# Autodesk Inventor assembly: 車体
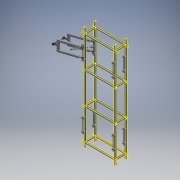
[picture p0: Inventor's stored thumbnail of the model, 180x180]
Saved by Autodesk Inventor 2018 (Build 220112000, 112)
## iProperties
Created: 2017-09-11
Part Number: 車体
Material: 一般
Document SubType Name: Assembly
Designer: mura5
Author: mura5
## Documents named in this file (8)
- C:\Users\Kenta\Documents\workspace\rbbr\cart\シャーシ改でアッカーマン検討\車体.iam
- C:\Users\Kenta\Documents\workspace\rbbr\cart\シャーシ改でアッカーマン検討\Pipe1.ipt
- C:\Users\Kenta\Documents\workspace\rbbr\cart\シャーシ改でアッカーマン検討\Pipe2.ipt
- C:\Users\Kenta\Documents\workspace\rbbr\cart\シャーシ改でアッカーマン検討\Pipe3.ipt
- C:\Users\Kenta\Documents\workspace\rbbr\cart\シャーシ改でアッカーマン検討\Pipe4.ipt
- C:\Users\Kenta\Documents\workspace\rbbr\cart\シャーシ\飛び出す奴上.iam
- C:\Users\Kenta\Documents\workspace\rbbr\cart\A.iam
- C:\Users\Kenta\Documents\workspace\rbbr\cart\スプリング.iam
## Components (31 placed, 7 different names)
1. Pipe1:1 — 回転:1, 角度:1, 回転:3, 角度:3, メイト:1, フラッシュ:1, フラッシュ:2, メイト:3, メイト:13, メイト:14, メイト:16, フラッシュ:5, メイト:18, フラッシュ:10, メイト:20, メイト:30, メイト:43, 角度:9
2. Pipe2:1 — 回転:1, 回転:2, 角度:1, 角度:2, メイト:2, フラッシュ:8, フラッシュ:9, 角度:5, メイト:31, メイト:37
3. Pipe1:2 — 回転:2, 角度:2, メイト:7, メイト:10, メイト:12, フラッシュ:7, メイト:17, メイト:35, 角度:7, メイト:45, 角度:11
4. Pipe2:2 — 回転:3, 角度:3, メイト:4, メイト:5, メイト:6, メイト:8, フラッシュ:12, メイト:48, メイト:50
5. Pipe3:1 — メイト:1, フラッシュ:1, メイト:2, メイト:11, フラッシュ:4, フラッシュ:6
6. Pipe3:2 — フラッシュ:2, メイト:3, メイト:4, メイト:9, フラッシュ:3, メイト:15
7. Pipe4:1 — メイト:5, フラッシュ:11, メイト:19, メイト:20, フラッシュ:12, フラッシュ:13
8. Pipe4:2 — メイト:6, メイト:7, メイト:8
9. Pipe4:3 — メイト:13, メイト:14, メイト:15
10. Pipe4:4 — メイト:16, フラッシュ:5, フラッシュ:6
11. Pipe4:5 — メイト:11, メイト:12, フラッシュ:4, フラッシュ:15
12. Pipe4:6 — メイト:9, メイト:10, フラッシュ:3, フラッシュ:16
13. Pipe4:7 — メイト:18, フラッシュ:9, フラッシュ:10
14. Pipe4:8 — フラッシュ:7, フラッシュ:8, メイト:17
15. Pipe1:3 — フラッシュ:11, メイト:19, 回転:4, メイト:21, メイト:28, 角度:4, メイト:46, 角度:8
16. Pipe1:4 — 回転:5, フラッシュ:14, 回転:6, メイト:22, メイト:23, メイト:24, メイト:26, メイト:27, メイト:34, 角度:6, メイト:44, 角度:10
17. Pipe2:3 — 回転:4, メイト:21, フラッシュ:13, 回転:5, フラッシュ:14, メイト:47, メイト:49
18. Pipe2:4 — 回転:6, メイト:22, メイト:29, メイト:36
19. Pipe3:3 — メイト:23, メイト:24, フラッシュ:15
20. Pipe3:4 — メイト:26, フラッシュ:16, メイト:27
21. 飛び出す奴上:1 [sub-assembly] — メイト:28, 角度:4, メイト:29, 円柱状:8, メイト:38, 回転:7
22. 飛び出す奴上:2 [sub-assembly] — メイト:30, 角度:5, メイト:31, 円柱状:9, メイト:39
23. 飛び出す奴上:3 [sub-assembly] — メイト:34, 角度:6, メイト:36
24. 飛び出す奴上:4 [sub-assembly] — メイト:35, 角度:7, メイト:37
25. A:1 [sub-assembly] — 円柱状:8, メイト:38, メイト:40, メイト:41
26. A:2 [sub-assembly] — 円柱状:9, メイト:39, メイト:40, メイト:41, メイト:51
27. 飛び出す奴上:5 [sub-assembly] — メイト:46, 角度:8, メイト:47
28. 飛び出す奴上:6 [sub-assembly] — メイト:43, 角度:9, メイト:48
29. 飛び出す奴上:7 [sub-assembly] — メイト:44, 角度:10, メイト:49
30. 飛び出す奴上:8 [sub-assembly] — メイト:45, 角度:11, メイト:50
31. スプリング:1 [sub-assembly] — 回転:7, メイト:51
## Relationships (83: Mate 47, Flush 16, Angle 11, RevoluteJoint 7, CylindricalJoint 2)
- 回転:1 [RevoluteJoint]: Pipe1:1 ↔ Pipe2:1
- 回転:2 [RevoluteJoint]: Pipe2:1 ↔ Pipe1:2
- 角度:1 [Angle] (90 deg): Pipe1:1 ↔ Pipe2:1
- 角度:2 [Angle] (90 deg): Pipe2:1 ↔ Pipe1:2
- 回転:3 [RevoluteJoint]: Pipe1:1 ↔ Pipe2:2
- 角度:3 [Angle] (90 deg): Pipe1:1 ↔ Pipe2:2
- メイト:1 [Mate]: Pipe1:1 ↔ Pipe3:1
- フラッシュ:1 [Flush]: Pipe1:1 ↔ Pipe3:1
- メイト:2 [Mate] (590.9333 mm): Pipe2:1 ↔ Pipe3:1
- フラッシュ:2 [Flush]: Pipe1:1 ↔ Pipe3:2
- メイト:3 [Mate]: Pipe1:1 ↔ Pipe3:2
- メイト:4 [Mate] (590.9333 mm): Pipe2:2 ↔ Pipe3:2
- メイト:5 [Mate]: Pipe2:2 ↔ Pipe4:1
- メイト:6 [Mate]: Pipe2:2 ↔ Pipe4:2
- メイト:7 [Mate]: Pipe1:2 ↔ Pipe4:2
- メイト:8 [Mate]: Pipe2:2 ↔ Pipe4:2
- メイト:9 [Mate]: Pipe3:2 ↔ Pipe4:6
- メイト:10 [Mate]: Pipe1:2 ↔ Pipe4:6
- フラッシュ:3 [Flush]: Pipe3:2 ↔ Pipe4:6
- メイト:11 [Mate]: Pipe3:1 ↔ Pipe4:5
- メイト:12 [Mate]: Pipe1:2 ↔ Pipe4:5
- フラッシュ:4 [Flush]: Pipe3:1 ↔ Pipe4:5
- メイト:13 [Mate]: Pipe1:1 ↔ Pipe4:3
- メイト:14 [Mate]: Pipe1:1 ↔ Pipe4:3
- メイト:15 [Mate]: Pipe3:2 ↔ Pipe4:3
- メイト:16 [Mate]: Pipe1:1 ↔ Pipe4:4
- フラッシュ:5 [Flush]: Pipe1:1 ↔ Pipe4:4
- フラッシュ:6 [Flush]: Pipe3:1 ↔ Pipe4:4
- フラッシュ:7 [Flush]: Pipe1:2 ↔ Pipe4:8
- フラッシュ:8 [Flush]: Pipe2:1 ↔ Pipe4:8
- メイト:17 [Mate]: Pipe1:2 ↔ Pipe4:8
- メイト:18 [Mate]: Pipe1:1 ↔ Pipe4:7
- フラッシュ:9 [Flush]: Pipe2:1 ↔ Pipe4:7
- フラッシュ:10 [Flush]: Pipe1:1 ↔ Pipe4:7
- フラッシュ:11 [Flush]: Pipe4:1 ↔ Pipe1:3
- メイト:19 [Mate]: Pipe4:1 ↔ Pipe1:3
- メイト:20 [Mate]: Pipe1:1 ↔ Pipe4:1
- フラッシュ:12 [Flush]: Pipe2:2 ↔ Pipe4:1
- 回転:4 [RevoluteJoint]: Pipe1:3 ↔ Pipe2:3
- メイト:21 [Mate]: Pipe1:3 ↔ Pipe2:3
- フラッシュ:13 [Flush]: Pipe4:1 ↔ Pipe2:3
- 回転:5 [RevoluteJoint]: Pipe1:4 ↔ Pipe2:3
- フラッシュ:14 [Flush]: Pipe1:4 ↔ Pipe2:3
- 回転:6 [RevoluteJoint]: Pipe1:4 ↔ Pipe2:4
- メイト:22 [Mate]: Pipe1:4 ↔ Pipe2:4
- メイト:23 [Mate]: Pipe1:4 ↔ Pipe3:3
- メイト:24 [Mate]: Pipe1:4 ↔ Pipe3:3
- フラッシュ:15 [Flush]: Pipe4:5 ↔ Pipe3:3
- メイト:26 [Mate]: Pipe1:4 ↔ Pipe3:4
- フラッシュ:16 [Flush]: Pipe4:6 ↔ Pipe3:4
- メイト:27 [Mate]: Pipe1:4 ↔ Pipe3:4
- メイト:28 [Mate]: Pipe1:3 ↔ 飛び出す奴上:1
- 角度:4 [Angle] (180 deg): Pipe1:3 ↔ 飛び出す奴上:1
- メイト:29 [Mate] (151.8665 mm): Pipe2:4 ↔ 飛び出す奴上:1
- メイト:30 [Mate]: Pipe1:1 ↔ 飛び出す奴上:2
- 角度:5 [Angle] (-90 deg): Pipe2:1 ↔ 飛び出す奴上:2
- メイト:31 [Mate] (151.8665 mm): Pipe2:1 ↔ 飛び出す奴上:2
- メイト:34 [Mate]: Pipe1:4 ↔ 飛び出す奴上:3
- メイト:35 [Mate]: Pipe1:2 ↔ 飛び出す奴上:4
- 角度:6 [Angle] (270 deg): Pipe1:4 ↔ 飛び出す奴上:3
- 角度:7 [Angle] (90 deg): Pipe1:2 ↔ 飛び出す奴上:4
- メイト:36 [Mate] (151.8665 mm): Pipe2:4 ↔ 飛び出す奴上:3
- メイト:37 [Mate] (151.8665 mm): Pipe2:1 ↔ 飛び出す奴上:4
- 円柱状:8 [CylindricalJoint]: 飛び出す奴上:1 ↔ A:1
- メイト:38 [Mate] (-2 mm): 飛び出す奴上:1 ↔ A:1
- 円柱状:9 [CylindricalJoint]: 飛び出す奴上:2 ↔ A:2
- メイト:39 [Mate] (-2 mm): 飛び出す奴上:2 ↔ A:2
- メイト:40 [Mate]: A:1 ↔ A:2
- メイト:41 [Mate] (83 mm): A:1 ↔ A:2
- メイト:43 [Mate]: Pipe1:1 ↔ 飛び出す奴上:6
- メイト:44 [Mate]: Pipe1:4 ↔ 飛び出す奴上:7
- メイト:45 [Mate]: Pipe1:2 ↔ 飛び出す奴上:8
- メイト:46 [Mate]: Pipe1:3 ↔ 飛び出す奴上:5
- 角度:8 [Angle] (90 deg): Pipe1:3 ↔ 飛び出す奴上:5
- 角度:9 [Angle] (90 deg): Pipe1:1 ↔ 飛び出す奴上:6
- 角度:10 [Angle] (-90 deg): Pipe1:4 ↔ 飛び出す奴上:7
- 角度:11 [Angle] (-90 deg): Pipe1:2 ↔ 飛び出す奴上:8
- メイト:47 [Mate] (151.8665 mm): Pipe2:3 ↔ 飛び出す奴上:5
- メイト:48 [Mate] (151.8665 mm): Pipe2:2 ↔ 飛び出す奴上:6
- メイト:49 [Mate] (151.8665 mm): Pipe2:3 ↔ 飛び出す奴上:7
- メイト:50 [Mate] (151.8665 mm): Pipe2:2 ↔ 飛び出す奴上:8
- 回転:7 [RevoluteJoint]: 飛び出す奴上:1 ↔ スプリング:1
- メイト:51 [Mate]: A:2 ↔ スプリング:1
